# Autodesk Inventor assembly: Main Assembly
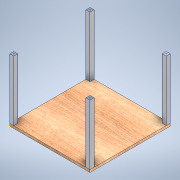
[picture p0: Inventor's stored thumbnail of the model, 180x180]
Saved by Autodesk Inventor 2020 (Build 240168000, 168)
## iProperties
Created: 2020-03-15
Part Number: Main Assembly
Document SubType Name: Assembly
Designer: Peter
Author: Peter
## Documents named in this file (4)
- C:\Users\Peter\Documents\Development\paragon-printer\Main Assembly.iam
- C:\Users\Peter\Documents\Development\paragon-printer\Stock\Base.ipt
- C:\Users\Peter\Documents\Development\paragon-printer\Stock\Tower.ipt
- C:\Users\Peter\Documents\Development\paragon-printer\Paragon Printer Parameters.xlsx
## Components (5 placed, 2 different names)
1. Base:1 — Mate:1, Mate:2, Mate:3, Mate:4, Mate:5
2. Tower:1 — Flush:3, Mate:4, Flush:6
3. Tower:2 — Flush:2, Flush:3, Mate:1, Mate:5, Flush:4
4. Tower:3 — Flush:1, Flush:2, Mate:3, Flush:4, Flush:5
5. Tower:4 — Flush:1, Mate:2, Flush:5, Flush:6
## Relationships (11: Flush 6, Mate 5)
- Flush:1: Tower:3 ↔ Tower:4
- Flush:2: Tower:2 ↔ Tower:3
- Flush:3: Tower:1 ↔ Tower:2
- Mate:1: Base:1 ↔ Tower:2
- Mate:2: Base:1 ↔ Tower:4
- Mate:3: Base:1 ↔ Tower:3
- Mate:4: Base:1 ↔ Tower:1
- Mate:5: Base:1 ↔ Tower:2
- Flush:4: Tower:2 ↔ Tower:3
- Flush:5: Tower:3 ↔ Tower:4
- Flush:6: Tower:1 ↔ Tower:4
## Named parameters: base_x_dim = 400 mm, base_y_dim = 400 mm, base_thickness = 12.7 mm, twenty = 20 mm, tower_height = 300 mm
